# Autodesk Inventor assembly: CC320b_Complete
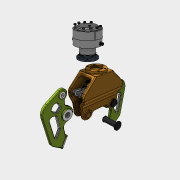
[picture p0: Inventor's stored thumbnail of the model, 180x180]
Saved by Autodesk Inventor 2020.1 (Build 241239000, 239)
## iProperties
Created: 2003-02-25
Part Number: CC320b_Complete
Document SubType Name: Assembly
Designer: Joe M
Engineer: Joe M
Control State: 0
Master: False
Checked Out: False
Shininess: 64.0
Length Units: 11269
Angle Units: 11279
Time Units: 11290
Mass Units: 11283
Length Display Precision: 3
Angle Display Precision: 2
Compacted: True
Density: 0.0
Volumn: 0.0
Area: 0.0
PropertySet Name: Model Information
Author: Joe M
## Documents named in this file (9)
- C:\Users\thom_tremblay\Desktop\Inventor ACP Data\Crusher Assembly.iam
- C:\Users\thom_tremblay\Desktop\Inventor ACP Data\Assemblies\Gripper.iam
- C:\Users\thom_tremblay\Desktop\Inventor ACP Data\Assemblies\BoltASM.iam
- C:\Users\thom_tremblay\Desktop\Inventor ACP Data\Parts\Layout_D_Complete.ipt
- C:\Users\thom_tremblay\Desktop\Inventor ACP Data\Content Center\local.DIN.19.282.1.ipt
- C:\Users\thom_tremblay\Desktop\Inventor ACP Data\Content Center\MyStandard.DIN.162.310.1.ipt
- C:\Users\thom_tremblay\Desktop\Inventor ACP Data\Parts\Crusher_Tooth.ipt
- C:\Users\thom_tremblay\Desktop\Inventor ACP Data\Actuator.iam
- C:\Users\thom_tremblay\Desktop\Inventor ACP Data\Assemblies\Hydro400.iam
## Components (21 placed, 8 different names)
1. Hydro400:1 [sub-assembly]
2. Gripper:1 [sub-assembly] — Mate:13, Mate:15, Mate:26
3. Gripper:2 [sub-assembly]
4. BoltASM:1 [sub-assembly] — Mate:13, Mate:15, Mate:26, Mate:56
5. BoltASM:2 [sub-assembly]
6. Layout_D_Complete:1 — Mate:53, Mate:56
7. Actuator:1 [sub-assembly]
8. Crusher_Tooth:1
9. Crusher_Tooth:2
10. DIN 125-1  B B 17:1 — Insert:5
11. DIN 933  (Regelgewinde) - ersetzt durch DIN EN 24 017 M16  x 40:1 — Insert:5
12. DIN 125-1  B B 17:2
13. DIN 933  (Regelgewinde) - ersetzt durch DIN EN 24 017 M16  x 40:2
14. DIN 125-1  B B 17:3
15. DIN 933  (Regelgewinde) - ersetzt durch DIN EN 24 017 M16  x 40:3
16. DIN 125-1  B B 17:4
17. DIN 933  (Regelgewinde) - ersetzt durch DIN EN 24 017 M16  x 40:4
18. DIN 125-1  B B 17:5
19. DIN 933  (Regelgewinde) - ersetzt durch DIN EN 24 017 M16  x 40:5
20. DIN 125-1  B B 17:6
21. DIN 933  (Regelgewinde) - ersetzt durch DIN EN 24 017 M16  x 40:6
## Component patterns: (6 elements, first: DIN 125-1  B B 17:1 + DIN 933  (Regelgewinde) - ersetzt durch DIN EN 24 017 M16  x 40:1)
## Relationships (12: Mate 8, Insert 2, Flush 1, Angle 1)
- Mate:13 (40 mm): Gripper:1 ↔ BoltASM:1
- Mate:15 (40 mm): Gripper:1 ↔ BoltASM:1
- [Mate]: Gripper:1 ↔ Actuator:1
- [Mate]: Gripper:1 ↔ Actuator:1
- Mate:26: Gripper:1 ↔ BoltASM:1
- [Mate]: Gripper:1 ↔ Actuator:1
- Mate:53: Layout_D_Complete:1
- [Flush]: Layout_D_Complete:1 ↔ Actuator:1
- [Angle] (0 deg): Layout_D_Complete:1 ↔ Actuator:1
- Mate:56: BoltASM:1 ↔ Layout_D_Complete:1
- Insert:5: DIN 125-1  B B 17:1 ↔ DIN 933  (Regelgewinde) - ersetzt durch DIN EN 24 017 M16  x 40:1
- [Insert]: Hydro400:1 ↔ DIN 125-1  B B 17:1
